# Autodesk Inventor assembly: wheel tip assembly
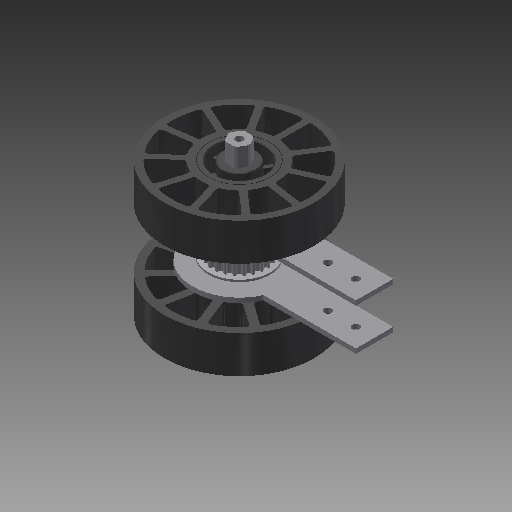
[picture p0: Inventor's stored thumbnail of the model, 512x512]
Saved by Autodesk Inventor 2018 (Build 220112000, 112)
## iProperties
Created: 2019-02-23
Part Number: wheel tip assembly
Document SubType Name: Assembly
Designer: s-2513225
Author: s-2513225
## Documents named in this file (6)
- C:\Users\s-2513225\Downloads\2019CAD-master\NEW NEW GRIPPER (feb 23)\wheel tip assembly.iam
- C:\Users\s-2513225\Downloads\2019CAD-master\NEW NEW GRIPPER (feb 23)\0_500_ID_x_1_125_OD_x_0_313_WD_Flanged_Bearing_217-2731.ipt
- C:\Users\s-2513225\Downloads\2019CAD-master\NEW NEW GRIPPER (feb 23)\1_2_Hex_x_0_201_ID_ThunderHex_Stock_18_217-4002.ipt
- \\studenthome\students\S-2513225\Inventor\24t_x_15mm_Wide_Aluminum_Pulley_HTD_5mm_1_2_Hex_217-4101.ipt
- C:\Users\s-2513225\Downloads\2019CAD-master\NEW NEW GRIPPER (feb 23)\am-3480 4IN 500Hex Bore Compliant Wheel.ipt
- C:\Users\s-2513225\Downloads\2019CAD-master\NEW NEW GRIPPER (feb 23)\wheel tip.ipt
## Components (8 placed, 5 different names)
1. 0_500_ID_x_1_125_OD_x_0_313_WD_Flanged_Bearing_217-2731:1 — Mate:1, Mate:2, Mate:7, Mate:14
2. 1_2_Hex_x_0_201_ID_ThunderHex_Stock_18_217-4002:1 — Mate:5, Mate:6, Mate:7, Mate:8, Mate:9, Mate:10, Mate:11, Mate:12
3. 24t_x_15mm_Wide_Aluminum_Pulley_HTD_5mm_1_2_Hex_217-4101:1 — Mate:8, Mate:9, Mate:13, Mate:14
4. am-3480 4IN 500Hex Bore Compliant Wheel:1 — Mate:5, Mate:6
5. wheel tip:1 — Mate:1, Mate:2, Flush:1, Flush:2
6. 0_500_ID_x_1_125_OD_x_0_313_WD_Flanged_Bearing_217-2731:2 — Mate:3, Mate:4, Mate:10, Mate:13
7. am-3480 4IN 500Hex Bore Compliant Wheel:2 — Mate:11, Mate:12
8. wheel tip:2 — Mate:3, Mate:4, Flush:1, Flush:2
## Relationships (16: Mate 14, Flush 2)
- Mate:1: 0_500_ID_x_1_125_OD_x_0_313_WD_Flanged_Bearing_217-2731:1 ↔ wheel tip:1
- Mate:2: 0_500_ID_x_1_125_OD_x_0_313_WD_Flanged_Bearing_217-2731:1 ↔ wheel tip:1
- Mate:3: 0_500_ID_x_1_125_OD_x_0_313_WD_Flanged_Bearing_217-2731:2 ↔ wheel tip:2
- Mate:4: 0_500_ID_x_1_125_OD_x_0_313_WD_Flanged_Bearing_217-2731:2 ↔ wheel tip:2
- Mate:5: 1_2_Hex_x_0_201_ID_ThunderHex_Stock_18_217-4002:1 ↔ am-3480 4IN 500Hex Bore Compliant Wheel:1
- Mate:6: 1_2_Hex_x_0_201_ID_ThunderHex_Stock_18_217-4002:1 ↔ am-3480 4IN 500Hex Bore Compliant Wheel:1
- Mate:7: 0_500_ID_x_1_125_OD_x_0_313_WD_Flanged_Bearing_217-2731:1 ↔ 1_2_Hex_x_0_201_ID_ThunderHex_Stock_18_217-4002:1
- Mate:8: 1_2_Hex_x_0_201_ID_ThunderHex_Stock_18_217-4002:1 ↔ 24t_x_15mm_Wide_Aluminum_Pulley_HTD_5mm_1_2_Hex_217-4101:1
- Mate:9: 1_2_Hex_x_0_201_ID_ThunderHex_Stock_18_217-4002:1 ↔ 24t_x_15mm_Wide_Aluminum_Pulley_HTD_5mm_1_2_Hex_217-4101:1
- Mate:10: 1_2_Hex_x_0_201_ID_ThunderHex_Stock_18_217-4002:1 ↔ 0_500_ID_x_1_125_OD_x_0_313_WD_Flanged_Bearing_217-2731:2
- Flush:1: wheel tip:1 ↔ wheel tip:2
- Flush:2: wheel tip:1 ↔ wheel tip:2
- Mate:11: 1_2_Hex_x_0_201_ID_ThunderHex_Stock_18_217-4002:1 ↔ am-3480 4IN 500Hex Bore Compliant Wheel:2
- Mate:12: 1_2_Hex_x_0_201_ID_ThunderHex_Stock_18_217-4002:1 ↔ am-3480 4IN 500Hex Bore Compliant Wheel:2
- Mate:13: 24t_x_15mm_Wide_Aluminum_Pulley_HTD_5mm_1_2_Hex_217-4101:1 ↔ 0_500_ID_x_1_125_OD_x_0_313_WD_Flanged_Bearing_217-2731:2
- Mate:14: 0_500_ID_x_1_125_OD_x_0_313_WD_Flanged_Bearing_217-2731:1 ↔ 24t_x_15mm_Wide_Aluminum_Pulley_HTD_5mm_1_2_Hex_217-4101:1
